# Autodesk Inventor assembly: HopperAssembly42inch_v5
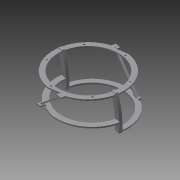
[picture p0: Inventor's stored thumbnail of the model, 180x180]
Saved by Autodesk Inventor 2013 (Build 170138000, 138)
## iProperties
Created: 2013-01-17
Part Number: HopperAssembly42inch_v5
Document SubType Name: Assembly
Designer: twsass
Author: twsass
## Documents named in this file (7)
- E:\Robotics\Hopper\HopperAssembly42inch_v5.iam
- E:\Robotics\Hopper\TopHoopSection_v4.ipt
- E:\Robotics\Hopper\HopperFrontSupport_v2.ipt
- E:\Robotics\Hopper\BottomHoop_v1.ipt
- E:\Robotics\Hopper\MiddleHoop.ipt
- E:\Robotics\Hopper\1Piecelongsupport_v1.ipt
- E:\Robotics\Hopper\1Pieceshortsupport_v1.ipt
## Components (8 placed, 6 different names)
1. TopHoopSection_v4:1 — Mate:113, Mate:114, Mate:115
2. HopperFrontSupport_v2:2 — Mate:78, Mate:79, Mate:80, Mate:107, Mate:108, Mate:109, Mate:116, Mate:117, Mate:118
3. TopHoopSection_v4:2 — Mate:116, Mate:117, Mate:118
4. BottomHoop_v1:1 — Mate:64, Mate:65, Mate:66, Mate:78, Mate:79, Mate:80, Mate:87, Mate:119, Mate:120, Mate:121
5. MiddleHoop:1 — Mate:107, Mate:108, Mate:109, Mate:145, Mate:146, Mate:147, Mate:148, Mate:149
6. HopperFrontSupport_v2:3 — Mate:64, Mate:65, Mate:66, Mate:113, Mate:114, Mate:115
7. 1Piecelongsupport_v1:1 — Mate:87, Mate:119, Mate:120, Mate:121
8. 1Pieceshortsupport_v1:1 — Mate:145, Mate:146, Mate:147, Mate:148, Mate:149
## Relationships (24: Mate 24)
- Mate:64: BottomHoop_v1:1 ↔ HopperFrontSupport_v2:3
- Mate:65: BottomHoop_v1:1 ↔ HopperFrontSupport_v2:3
- Mate:66: BottomHoop_v1:1 ↔ HopperFrontSupport_v2:3
- Mate:78: HopperFrontSupport_v2:2 ↔ BottomHoop_v1:1
- Mate:79: HopperFrontSupport_v2:2 ↔ BottomHoop_v1:1
- Mate:80: HopperFrontSupport_v2:2 ↔ BottomHoop_v1:1
- Mate:87: BottomHoop_v1:1 ↔ 1Piecelongsupport_v1:1
- Mate:107: HopperFrontSupport_v2:2 ↔ MiddleHoop:1
- Mate:108: HopperFrontSupport_v2:2 ↔ MiddleHoop:1
- Mate:109: HopperFrontSupport_v2:2 ↔ MiddleHoop:1
- Mate:113: TopHoopSection_v4:1 ↔ HopperFrontSupport_v2:3
- Mate:114: TopHoopSection_v4:1 ↔ HopperFrontSupport_v2:3
- Mate:115: TopHoopSection_v4:1 ↔ HopperFrontSupport_v2:3
- Mate:116: HopperFrontSupport_v2:2 ↔ TopHoopSection_v4:2
- Mate:117: HopperFrontSupport_v2:2 ↔ TopHoopSection_v4:2
- Mate:118: HopperFrontSupport_v2:2 ↔ TopHoopSection_v4:2
- Mate:119: BottomHoop_v1:1 ↔ 1Piecelongsupport_v1:1
- Mate:120: BottomHoop_v1:1 ↔ 1Piecelongsupport_v1:1
- Mate:121: BottomHoop_v1:1 ↔ 1Piecelongsupport_v1:1
- Mate:145: MiddleHoop:1 ↔ 1Pieceshortsupport_v1:1
- Mate:146: MiddleHoop:1 ↔ 1Pieceshortsupport_v1:1
- Mate:147: MiddleHoop:1 ↔ 1Pieceshortsupport_v1:1
- Mate:148: MiddleHoop:1 ↔ 1Pieceshortsupport_v1:1
- Mate:149: MiddleHoop:1 ↔ 1Pieceshortsupport_v1:1
